# Autodesk Inventor assembly: POM_T5_25
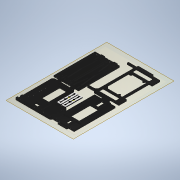
[picture p0: Inventor's stored thumbnail of the model, 180x180]
Saved by Autodesk Inventor 2020 (Build 240168000, 168)
## iProperties
Created: 2021-08-27
Part Number: POM_T5_25
Document SubType Name: Assembly
Designer: Masato
Author: Masato
## Documents named in this file (8)
- C:\Users\ptcga\OneDrive\ドキュメント\SUSTAINA-OP\Cam\POM_T5_25.iam
- C:\Users\ptcga\OneDrive\ドキュメント\SUSTAINA-OP\Cam\DisposableBoard.ipt
- C:\Users\ptcga\OneDrive\ドキュメント\SUSTAINA-OP\UpperBody\Cockpit\Cockpit_battery_bottom_frame.ipt
- C:\Users\ptcga\OneDrive\ドキュメント\SUSTAINA-OP\UpperBody\Cockpit\Cockpit_carrier_board_frame.ipt
- C:\Users\ptcga\OneDrive\ドキュメント\SUSTAINA-OP\UpperBody\Cockpit\Cockpit_side_frame_MIR.ipt
- C:\Users\ptcga\OneDrive\ドキュメント\SUSTAINA-OP\UpperBody\Cockpit\Cockpit_battery_front_frame.ipt
- C:\Users\ptcga\OneDrive\ドキュメント\SUSTAINA-OP\UpperBody\Cockpit\Cockpit_back_frame.ipt
- C:\Users\ptcga\OneDrive\ドキュメント\SUSTAINA-OP\Jig\Camera_side_frame_Jig.ipt
## Components (8 placed, 7 different names)
1. DisposableBoard:1 — メイト:2, メイト:1, フラッシュ:1, フラッシュ:2, メイト:4, メイト:5, メイト:6, メイト:7, フラッシュ:3, フラッシュ:4, フラッシュ:5, メイト:11, フラッシュ:8, メイト:14
2. Cockpit_side_frame_MIR:1 — メイト:4, フラッシュ:4, フラッシュ:5, メイト:10, メイト:12, フラッシュ:7, メイト:15, メイト:16
3. Cockpit_battery_bottom_frame:1 — メイト:5, フラッシュ:3, メイト:8, メイト:10, フラッシュ:6
4. Cockpit_battery_front_frame:1 — メイト:6, メイト:8, フラッシュ:6
5. Cockpit_carrier_board_frame:1 — メイト:7, メイト:13, フラッシュ:8
6. Cockpit_back_frame:1 — メイト:11, メイト:12, フラッシュ:7, メイト:13
7. Camera_side_frame_Jig:1 — メイト:14, メイト:15, メイト:16
8. Camera_side_frame_Jig:2
## Component patterns: (2 elements, first: Camera_side_frame_Jig:1)
## Relationships (22: Mate 14, Flush 8)
- メイト:2 [Mate]: DisposableBoard:1
- メイト:1 [Mate]: DisposableBoard:1
- フラッシュ:1 [Flush]: DisposableBoard:1
- フラッシュ:2 [Flush]: DisposableBoard:1
- メイト:4 [Mate]: DisposableBoard:1 ↔ Cockpit_side_frame_MIR:1
- メイト:5 [Mate]: DisposableBoard:1 ↔ Cockpit_battery_bottom_frame:1
- メイト:6 [Mate]: DisposableBoard:1 ↔ Cockpit_battery_front_frame:1
- メイト:7 [Mate]: DisposableBoard:1 ↔ Cockpit_carrier_board_frame:1
- フラッシュ:3 [Flush] (2 mm): DisposableBoard:1 ↔ Cockpit_battery_bottom_frame:1
- メイト:8 [Mate] (2.5 mm): Cockpit_battery_bottom_frame:1 ↔ Cockpit_battery_front_frame:1
- フラッシュ:4 [Flush] (2 mm): DisposableBoard:1 ↔ Cockpit_side_frame_MIR:1
- フラッシュ:5 [Flush] (2 mm): DisposableBoard:1 ↔ Cockpit_side_frame_MIR:1
- メイト:10 [Mate] (2.5 mm): Cockpit_side_frame_MIR:1 ↔ Cockpit_battery_bottom_frame:1
- フラッシュ:6 [Flush]: Cockpit_battery_bottom_frame:1 ↔ Cockpit_battery_front_frame:1
- メイト:11 [Mate]: DisposableBoard:1 ↔ Cockpit_back_frame:1
- メイト:12 [Mate] (2.5 mm): Cockpit_side_frame_MIR:1 ↔ Cockpit_back_frame:1
- フラッシュ:7 [Flush]: Cockpit_side_frame_MIR:1 ↔ Cockpit_back_frame:1
- メイト:13 [Mate] (2.5 mm): Cockpit_carrier_board_frame:1 ↔ Cockpit_back_frame:1
- フラッシュ:8 [Flush] (10 mm): DisposableBoard:1 ↔ Cockpit_carrier_board_frame:1
- メイト:14 [Mate]: DisposableBoard:1 ↔ Camera_side_frame_Jig:1
- メイト:15 [Mate] (2.5 mm): Cockpit_side_frame_MIR:1 ↔ Camera_side_frame_Jig:1
- メイト:16 [Mate] (2.5 mm): Cockpit_side_frame_MIR:1 ↔ Camera_side_frame_Jig:1
